# Autodesk Inventor assembly: 217-2428-031 Rev1
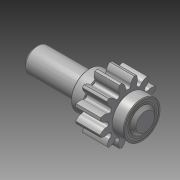
[picture p0: Inventor's stored thumbnail of the model, 180x180]
Saved by Autodesk Inventor 2014 SP1 (Build 180222100, 222)
## iProperties
Created: 2014-01-07
Part Number: 217-2428-031 Rev1
Document SubType Name: Assembly
Designer: Andrew Toennies
Mass: 13.0661 g
Surface Area: 29.6336 cm^2
Volume: 1.66447 cm^3
Density: 7.85 g/cm^3
Author: Andrew Toennies
## Documents named in this file (4)
- C:\Users\Moses\Documents\Inventor\Robot\Constrained 2 Speed Ball Shifter\217-2428-031 Rev1.iam
- C:\Users\Moses\Documents\Inventor\Robot\Constrained 2 Speed Ball Shifter\PINL-0250-1125-S.ipt
- C:\Users\Moses\Documents\Inventor\Robot\Constrained 2 Speed Ball Shifter\217-2788_57155K375.ipt
- C:\Users\Moses\Documents\Inventor\Robot\Constrained 2 Speed Ball Shifter\217-2428-017 Rev2.ipt
## Components (4 placed, 4 different names)
1. PINL-0250-1125-S_73 — Flush:1, Mate:1, Mate:2, Flush:2, Mate:3
2. 217-2788_57155K375_74 — Flush:1, Mate:1
3. 217-2788_57155K375_75 — Mate:2, Mate:4
4. 217-2428-017 Rev2_76 — Flush:2, Mate:3, Mate:4
## Relationships (6: Mate 4, Flush 2)
- Flush:1 (-0.762 mm): PINL-0250-1125-S_73 ↔ 217-2788_57155K375_74
- Mate:1: PINL-0250-1125-S_73 ↔ 217-2788_57155K375_74
- Mate:2: PINL-0250-1125-S_73 ↔ 217-2788_57155K375_75
- Flush:2 (4.445 mm): PINL-0250-1125-S_73 ↔ 217-2428-017 Rev2_76
- Mate:3: PINL-0250-1125-S_73 ↔ 217-2428-017 Rev2_76
- Mate:4 (0.508 mm): 217-2788_57155K375_75 ↔ 217-2428-017 Rev2_76
